# Autodesk Inventor assembly: зажим
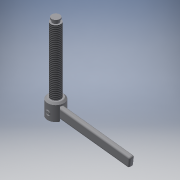
[picture p0: Inventor's stored thumbnail of the model, 180x180]
Saved by Autodesk Inventor 2019 (Build 230136000, 136)
## iProperties
Created: 2019-04-30
Part Number: зажим
Material: Типовые
Document SubType Name: Assembly
Designer: BarmanKaktus
Author: BarmanKaktus
## Documents named in this file (4)
- E:\Автодоска\файлы из доски\мясорубка\зажим.iam
- E:\Автодоска\файлы из доски\мясорубка\ручка.ipt
- E:\Автодоска\файлы из доски\мясорубка\крепёж.ipt
- E:\Автодоска\файлы из доски\мясорубка\штифт.ipt
## Components (3 placed, 3 different names)
1. ручка:1 — Совмещение:1, Совмещение:2
2. крепёж:1 — Совмещение:1, Совмещение:2, Совмещение:3, Совмещение:4
3. штифт:1 — Совмещение:3, Совмещение:4
## Relationships (4: Mate 4)
- Совмещение:1 [Mate]: ручка:1 ↔ крепёж:1
- Совмещение:2 [Mate] (0.5 mm): ручка:1 ↔ крепёж:1
- Совмещение:3 [Mate]: крепёж:1 ↔ штифт:1
- Совмещение:4 [Mate] (5 mm): крепёж:1 ↔ штифт:1
